# Autodesk Inventor assembly: 足全体
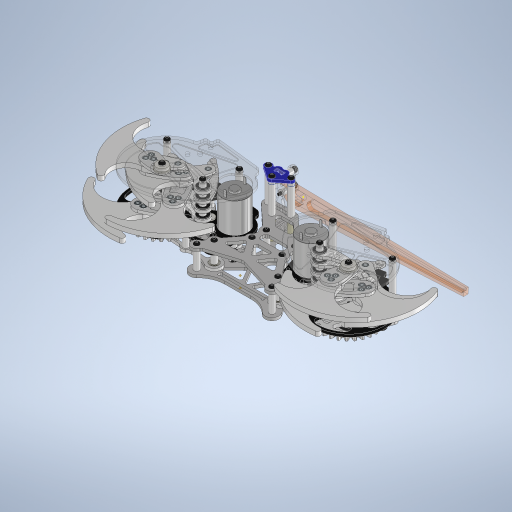
[picture p0: Inventor's stored thumbnail of the model, 512x512]
Saved by Autodesk Inventor 2023 (Build 270158000, 158)
## iProperties
Created: 2022-01-30
Part Number: 足全体
Document SubType Name: Assembly
Designer: acps
Mass: 767.98 g
Surface Area: 2765.24 cm^2
Volume: 318.532 cm^3
Density: 2.411 g/cm^3
Author: acps
## Documents named in this file (20)
- C:\Users\muzho\Documents\srdc\srdc_2\脚\足全体.iam
- C:\Users\muzho\Documents\srdc\srdc_2\脚\足ユニット.iam
- C:\Users\muzho\Documents\srdc\srdc_2\スペーサ\l23.ipt
- C:\Users\muzho\Documents\srdc\srdc_2\タミヤダンパー1.iam
- C:\Users\muzho\Documents\srdc\srdc_2\スペーサ\l10.ipt
- C:\Users\muzho\Documents\srdc\srdc_2\スペーサ\l7.ipt
- C:\Users\muzho\Documents\srdc\srdc_2\スペーサ\l3.ipt
- C:\Users\muzho\Documents\srdc\srdc_2\スペーサ\l23_peak.ipt
- C:\Users\muzho\Documents\srdc\srdc_2\スペーサ\l30.ipt
- C:\Users\muzho\Documents\srdc\srdc_2\脚\ウィング関連\足 横wing下板 .ipt
- C:\Users\muzho\Documents\srdc\srdc_2\脚\ウィング関連\足 横wing固定用外フレーム.ipt
- C:\Users\muzho\Documents\srdc\srdc_2\スペーサ\l12.ipt
- C:\Users\muzho\Documents\srdc\srdc_2\脚\ウィング関連\横wing 押さえ.ipt
- C:\Users\muzho\Documents\srdc\srdc_2\脚\ウィング関連\横wing _MIR.ipt
- C:\Users\muzho\Documents\srdc\srdc_2\脚\外中間ユニット.ipt
- C:\Users\muzho\Documents\srdc\srdc_2\脚\内中間ユニット.ipt
- C:\Users\muzho\Documents\srdc\srdc_2\脚\MIR\足ユニット_MIR.iam
- C:\Users\muzho\Documents\srdc\srdc_2\ねじ\M3ボタンボルト8.ipt
- C:\Users\muzho\Documents\srdc\srdc_2\ねじ\M3ボタンボルト35.ipt
- C:\Users\muzho\Documents\srdc\srdc_2\ねじ\M3ボタンボルト18.ipt
## Components (57 placed, 19 different names)
1. 足ユニット:1 [sub-assembly] — 挿入:23, メイト:18
2. l23:1 — 挿入:63, 挿入:65, メイト:24
3. l23:4 — メイト:18, メイト:19, メイト:20, 挿入:61
4. l23:7 — 挿入:62
5. l23:8 — 挿入:64
6. タミヤダンパー1:1 [sub-assembly] — 挿入:24, 挿入:53
7. l10:1 — 挿入:23, 挿入:24
8. l7:1 — 挿入:52, 挿入:53
9. l3:1 — 挿入:43
10. l3:2 — 挿入:42, 挿入:45
11. l3:3 — 挿入:44, メイト:11, 挿入:48
12. l23_peak:1 — 挿入:58
13. l23_peak:2 — 挿入:55
14. l23_peak:3 — 挿入:60
15. l30:1 — 挿入:44, 挿入:56
16. l30:2 — 挿入:42, 挿入:57
17. l30:3 — 挿入:43, 挿入:59
18. 足 横wing下板 :1 — 挿入:49, 挿入:50, メイト:17, メイト:22, メイト:23, フラッシュ:1
19. 足 横wing固定用外フレーム:1 — メイト:11, 挿入:45, 挿入:48, 挿入:82, 挿入:83, 挿入:84
20. l12:1 — 挿入:50, 挿入:51, メイト:16
21. l12:2 — 挿入:49, メイト:14, メイト:15
22. 横wing 押さえ:1 — メイト:14, 挿入:51, 挿入:96, 挿入:97
23. 横wing _MIR:1 — メイト:15, メイト:16, メイト:17
24. 外中間ユニット:1 — メイト:19, メイト:21, 挿入:56, 挿入:57, 挿入:59, 挿入:60, 挿入:61, 挿入:65, 挿入:85, 挿入:86, 挿入:87, 挿入:88, 挿入:89, 挿入:90, 挿入:91, 挿入:92
25. 内中間ユニット:1 — メイト:20, メイト:21, 挿入:52, 挿入:55, メイト:22, メイト:23, フラッシュ:1, 挿入:58, 挿入:62, 挿入:63, 挿入:64, 挿入:66, 挿入:67, 挿入:68, 挿入:69, 挿入:70, 挿入:74, 挿入:75, 挿入:76, 挿入:77, 挿入:78, 挿入:79, 挿入:80, 挿入:81, 挿入:93, 挿入:94, 挿入:95
26. l23:9 — 挿入:69
27. l23:10 — 挿入:68
28. l23:11 — 挿入:67
29. l23:12 — 挿入:66
30. 足ユニット_MIR:1 [sub-assembly] — メイト:24, 挿入:71
31. l7:2 — 挿入:70, メイト:25, 挿入:73
32. l10:2 — 挿入:71, メイト:26, 挿入:72
33. タミヤダンパー1:2 [sub-assembly] — メイト:25, メイト:26, 挿入:72, 挿入:73
34. M3ボタンボルト8:1 — 挿入:80
35. M3ボタンボルト8:2 — 挿入:79
36. M3ボタンボルト8:3 — 挿入:77
37. M3ボタンボルト8:4 — 挿入:75
38. M3ボタンボルト8:5 — 挿入:76
39. M3ボタンボルト8:6 — 挿入:74
40. M3ボタンボルト8:7 — 挿入:78
41. M3ボタンボルト8:8 — 挿入:85
42. M3ボタンボルト8:9 — 挿入:81
43. M3ボタンボルト8:10 — 挿入:82
44. M3ボタンボルト8:11 — 挿入:87
45. M3ボタンボルト8:12 — 挿入:86
46. M3ボタンボルト8:13 — 挿入:84
47. M3ボタンボルト8:14 — 挿入:88
48. M3ボタンボルト8:15 — 挿入:83
49. M3ボタンボルト8:16 — 挿入:91
50. M3ボタンボルト8:17 — 挿入:90
51. M3ボタンボルト8:18 — 挿入:89
52. M3ボタンボルト8:19 — 挿入:92
53. M3ボタンボルト35:1 — 挿入:94
54. M3ボタンボルト35:2 — 挿入:95
55. M3ボタンボルト35:3 — 挿入:93
56. M3ボタンボルト18:1 — 挿入:97
57. M3ボタンボルト18:2 — 挿入:96
## Relationships (70: Insert 55, Mate 14, Flush 1)
- 挿入:23 [Insert]: 足ユニット:1 ↔ l10:1
- 挿入:24 [Insert]: タミヤダンパー1:1 ↔ l10:1
- 挿入:42 [Insert]: l3:2 ↔ l30:2
- 挿入:43 [Insert]: l3:1 ↔ l30:3
- 挿入:44 [Insert]: l3:3 ↔ l30:1
- メイト:11 [Mate]: l3:3 ↔ 足 横wing固定用外フレーム:1
- 挿入:45 [Insert]: l3:2 ↔ 足 横wing固定用外フレーム:1
- 挿入:48 [Insert]: l3:3 ↔ 足 横wing固定用外フレーム:1
- 挿入:49 [Insert]: 足 横wing下板 :1 ↔ l12:2
- 挿入:50 [Insert]: 足 横wing下板 :1 ↔ l12:1
- メイト:14 [Mate]: l12:2 ↔ 横wing 押さえ:1
- 挿入:51 [Insert]: l12:1 ↔ 横wing 押さえ:1
- メイト:15 [Mate]: l12:2 ↔ 横wing _MIR:1
- メイト:16 [Mate]: l12:1 ↔ 横wing _MIR:1
- メイト:17 [Mate] (5 mm): 足 横wing下板 :1 ↔ 横wing _MIR:1
- メイト:18 [Mate]: 足ユニット:1 ↔ l23:4
- メイト:19 [Mate]: l23:4 ↔ 外中間ユニット:1
- メイト:20 [Mate]: l23:4 ↔ 内中間ユニット:1
- メイト:21 [Mate]: 外中間ユニット:1 ↔ 内中間ユニット:1
- 挿入:52 [Insert]: l7:1 ↔ 内中間ユニット:1
- 挿入:53 [Insert]: タミヤダンパー1:1 ↔ l7:1
- 挿入:55 [Insert]: l23_peak:2 ↔ 内中間ユニット:1
- メイト:22 [Mate]: 足 横wing下板 :1 ↔ 内中間ユニット:1
- メイト:23 [Mate]: 足 横wing下板 :1 ↔ 内中間ユニット:1
- フラッシュ:1 [Flush]: 足 横wing下板 :1 ↔ 内中間ユニット:1
- 挿入:56 [Insert]: l30:1 ↔ 外中間ユニット:1
- 挿入:57 [Insert]: l30:2 ↔ 外中間ユニット:1
- 挿入:58 [Insert]: l23_peak:1 ↔ 内中間ユニット:1
- 挿入:59 [Insert]: l30:3 ↔ 外中間ユニット:1
- 挿入:60 [Insert]: l23_peak:3 ↔ 外中間ユニット:1
- 挿入:61 [Insert]: l23:4 ↔ 外中間ユニット:1
- 挿入:62 [Insert]: l23:7 ↔ 内中間ユニット:1
- 挿入:63 [Insert]: l23:1 ↔ 内中間ユニット:1
- 挿入:64 [Insert]: l23:8 ↔ 内中間ユニット:1
- 挿入:65 [Insert]: l23:1 ↔ 外中間ユニット:1
- 挿入:66 [Insert]: 内中間ユニット:1 ↔ l23:12
- 挿入:67 [Insert]: 内中間ユニット:1 ↔ l23:11
- 挿入:68 [Insert]: 内中間ユニット:1 ↔ l23:10
- 挿入:69 [Insert]: 内中間ユニット:1 ↔ l23:9
- メイト:24 [Mate]: l23:1 ↔ 足ユニット_MIR:1
- 挿入:70 [Insert]: 内中間ユニット:1 ↔ l7:2
- 挿入:71 [Insert]: 足ユニット_MIR:1 ↔ l10:2
- メイト:25 [Mate]: l7:2 ↔ タミヤダンパー1:2
- メイト:26 [Mate]: l10:2 ↔ タミヤダンパー1:2
- 挿入:72 [Insert]: l10:2 ↔ タミヤダンパー1:2
- 挿入:73 [Insert]: l7:2 ↔ タミヤダンパー1:2
- 挿入:74 [Insert]: 内中間ユニット:1 ↔ M3ボタンボルト8:6
- 挿入:75 [Insert]: 内中間ユニット:1 ↔ M3ボタンボルト8:4
- 挿入:76 [Insert]: 内中間ユニット:1 ↔ M3ボタンボルト8:5
- 挿入:77 [Insert]: 内中間ユニット:1 ↔ M3ボタンボルト8:3
- 挿入:78 [Insert]: 内中間ユニット:1 ↔ M3ボタンボルト8:7
- 挿入:79 [Insert]: 内中間ユニット:1 ↔ M3ボタンボルト8:2
- 挿入:80 [Insert]: 内中間ユニット:1 ↔ M3ボタンボルト8:1
- 挿入:81 [Insert]: 内中間ユニット:1 ↔ M3ボタンボルト8:9
- 挿入:82 [Insert]: 足 横wing固定用外フレーム:1 ↔ M3ボタンボルト8:10
- 挿入:83 [Insert]: 足 横wing固定用外フレーム:1 ↔ M3ボタンボルト8:15
- 挿入:84 [Insert]: 足 横wing固定用外フレーム:1 ↔ M3ボタンボルト8:13
- 挿入:85 [Insert]: 外中間ユニット:1 ↔ M3ボタンボルト8:8
- 挿入:86 [Insert]: 外中間ユニット:1 ↔ M3ボタンボルト8:12
- 挿入:87 [Insert]: 外中間ユニット:1 ↔ M3ボタンボルト8:11
- 挿入:88 [Insert]: 外中間ユニット:1 ↔ M3ボタンボルト8:14
- 挿入:89 [Insert]: 外中間ユニット:1 ↔ M3ボタンボルト8:18
- 挿入:90 [Insert]: 外中間ユニット:1 ↔ M3ボタンボルト8:17
- 挿入:91 [Insert]: 外中間ユニット:1 ↔ M3ボタンボルト8:16
- 挿入:92 [Insert]: 外中間ユニット:1 ↔ M3ボタンボルト8:19
- 挿入:93 [Insert]: 内中間ユニット:1 ↔ M3ボタンボルト35:3
- 挿入:94 [Insert]: 内中間ユニット:1 ↔ M3ボタンボルト35:1
- 挿入:95 [Insert]: 内中間ユニット:1 ↔ M3ボタンボルト35:2
- 挿入:96 [Insert]: 横wing 押さえ:1 ↔ M3ボタンボルト18:2
- 挿入:97 [Insert]: 横wing 押さえ:1 ↔ M3ボタンボルト18:1
